# Autodesk Inventor assembly: Assembly1
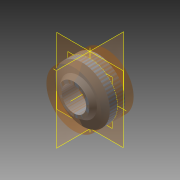
[picture p0: Inventor's stored thumbnail of the model, 180x180]
Saved by Autodesk Inventor 2018.2 (Build 222227000, 227)
## iProperties
Created: 2018-02-28
Part Number: Assembly1
Document SubType Name: Assembly
Designer: Rus
Author: Rus
## Documents named in this file (3)
- E:\Libraries\3D Objects\Longboard\Spacer and Rings\Assembly1.iam
- E:\Libraries\3D Objects\Longboard\Spacer and Rings\Spacer.ipt
- E:\Libraries\3D Objects\Longboard\Inside Wheels Limits\V0\Inside Wheel Limits.ipt
## Components (2 placed, 2 different names)
1. Spacer:1 — Angle:1, Tangent:1, Flush:1, Angle:2, Mate:1
2. Inside Wheel Limits:1 — Angle:1, Tangent:1, Flush:1, Angle:2, Mate:1
## Relationships (5: Angle 2, Tangent 1, Flush 1, Mate 1)
- Angle:1 (0 deg): Spacer:1 ↔ Inside Wheel Limits:1
- Tangent:1: Spacer:1 ↔ Inside Wheel Limits:1
- Flush:1: Spacer:1 ↔ Inside Wheel Limits:1
- Angle:2 (0 deg): Spacer:1 ↔ Inside Wheel Limits:1
- Mate:1: Spacer:1 ↔ Inside Wheel Limits:1
